# Autodesk Inventor assembly: Motor_plus_Rad
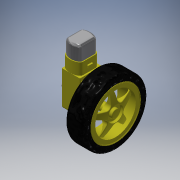
[picture p0: Inventor's stored thumbnail of the model, 180x180]
Saved by Autodesk Inventor 2017 SP1 (Build 210196100, 196)
## iProperties
Part Number: Motor_plus_Rad
Material: Generisch
Document SubType Name: Assembly
Designer: Alex
Author: Alex
## Documents named in this file (3)
- E:\Users\Alex\Documents\Inventor\Aktor\Motor\Motor_plus_Rad.iam
- E:\Users\Alex\Documents\Inventor\Aktor\Motor\Motor.ipt
- E:\Users\Alex\Documents\Inventor\Aktor\Motor\Rad.ipt
## Components (2 placed, 2 different names)
1. Motor:1 — Passend:1, Passend:2
2. Rad:1 — Passend:1, Passend:2
## Relationships (2: Mate 2)
- Passend:1 [Mate]: Motor:1 ↔ Rad:1
- Passend:2 [Mate]: Motor:1 ↔ Rad:1
